# Autodesk Inventor assembly: CLAW
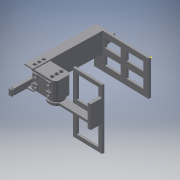
[picture p0: Inventor's stored thumbnail of the model, 180x180]
Saved by Autodesk Inventor 2016 (Build 200138000, 138)
## iProperties
Created: 2016-05-06
Part Number: CLAW
Document SubType Name: Assembly
Designer: mkepler
Author: mkepler
## Documents named in this file (6)
- C:\Users\mkepler\Google Drive\Michael Kepler\College\ECE\ECE 590\Project 3\Physical Design\Inventor Files\Claw\CLAW.iam
- C:\Users\mkepler\Google Drive\Michael Kepler\College\ECE\ECE 590\Project 3\Physical Design\Inventor Files\xl320Servo.ipt
- C:\Users\mkepler\Google Drive\Michael Kepler\College\ECE\ECE 590\Project 3\Physical Design\Inventor Files\Claw\GripperRight.ipt
- C:\Users\mkepler\Google Drive\Michael Kepler\College\ECE\ECE 590\Project 3\Physical Design\Inventor Files\Claw\GripperLeft.ipt
- C:\Users\mkepler\Google Drive\Michael Kepler\College\ECE\ECE 590\Project 3\Physical Design\Inventor Files\Claw\GripperLeftContact.ipt
- C:\Users\mkepler\Google Drive\Michael Kepler\College\ECE\ECE 590\Project 3\Physical Design\Inventor Files\Claw\ClawExtender.ipt
## Components (5 placed, 5 different names)
1. xl320Servo:1 — Insert:1, Insert:2, Insert:3, Insert:4
2. GripperRight:1 — Insert:1, Insert:2
3. GripperLeft:1 — Insert:3, Insert:4, Mate:1, Mate:2, Mate:4
4. GripperLeftContact:1 — Mate:1, Mate:2, Mate:4, Mate:5, Mate:6
5. ClawExtender:1 — Mate:5, Mate:6
## Relationships (9: Mate 5, Insert 4)
- Insert:1: xl320Servo:1 ↔ GripperRight:1
- Insert:2: xl320Servo:1 ↔ GripperRight:1
- Insert:3: xl320Servo:1 ↔ GripperLeft:1
- Insert:4: xl320Servo:1 ↔ GripperLeft:1
- Mate:1: GripperLeft:1 ↔ GripperLeftContact:1
- Mate:2: GripperLeft:1 ↔ GripperLeftContact:1
- Mate:4: GripperLeft:1 ↔ GripperLeftContact:1
- Mate:5: GripperLeftContact:1 ↔ ClawExtender:1
- Mate:6: GripperLeftContact:1 ↔ ClawExtender:1
